# Autodesk Inventor assembly: Functioning elevator (frame)
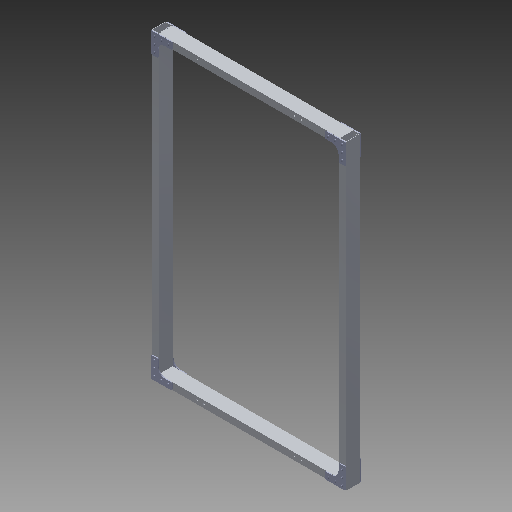
[picture p0: Inventor's stored thumbnail of the model, 512x512]
Saved by Autodesk Inventor 2019 (Build 230136000, 136)
## iProperties
Created: 2019-01-17
Part Number: Functioning elevator (frame)
Document SubType Name: Assembly
Designer: josh
Mass: 2454.62 g
Surface Area: 11117.3 cm^2
Volume: 909.118 cm^3
Density: 2.7 g/cm^3
Author: josh
## Documents named in this file (4)
- D:\Synthesis Robots\Epsilon\Epsilon elavator lift\Functioning elevator (frame).iam
- D:\Synthesis Robots\Epsilon\Epsilon elavator lift\Functioning elevator parts\Example Fixed Tube.ipt
- D:\Synthesis Robots\Epsilon\Epsilon elavator lift\Functioning elevator parts\Example Cross Frame Tube.ipt
- D:\Synthesis Robots\Epsilon\Epsilon elavator lift\Functioning elevator parts\am-3860 90 Gusset with Rivets.iam
## Components (12 placed, 3 different names)
1. Example Fixed Tube:1 — Flush:8, Mate:6, Flush:9, Flush:11, Flush:18, Flush:20, Flush:22, Mate:16
2. Example Fixed Tube:2 — Flush:2, Flush:3, Mate:2, Mate:3, Flush:5, Flush:6, Flush:7, Flush:13, Mate:9, Flush:16, Flush:17, Mate:15
3. Example Cross Frame Tube:1 — Flush:14, Flush:15, Mate:11, Mate:12, Flush:17, Flush:19, Mate:13, Flush:21, Mate:14, Mate:15, Mate:16
4. Example Cross Frame Tube:2 — Mate:1, Mate:2, Flush:4, Mate:4, Flush:8, Flush:10, Mate:7, Flush:12, Mate:8
5. am-3860 90 Gusset with Rivets:1 [sub-assembly] — Flush:13, Flush:14, Mate:9, Mate:11
6. am-3860 90 Gusset with Rivets:2 [sub-assembly] — Flush:15, Flush:16, Mate:12
7. am-3860 90 Gusset with Rivets:3 [sub-assembly] — Flush:18, Flush:21, Flush:22, Mate:14
8. am-3860 90 Gusset with Rivets:4 [sub-assembly] — Flush:19, Flush:20, Mate:13
9. am-3860 90 Gusset with Rivets:5 [sub-assembly] — Flush:3, Flush:6, Flush:7, Mate:4
10. am-3860 90 Gusset with Rivets:6 [sub-assembly] — Mate:1, Flush:2, Flush:4, Mate:3, Flush:5
11. am-3860 90 Gusset with Rivets:7 [sub-assembly] — Mate:6, Flush:9, Flush:10, Mate:7
12. am-3860 90 Gusset with Rivets:8 [sub-assembly] — Flush:11, Flush:12, Mate:8
## Relationships (35: Flush 21, Mate 14)
- Mate:1: Example Cross Frame Tube:2 ↔ am-3860 90 Gusset with Rivets:6
- Flush:2: Example Fixed Tube:2 ↔ am-3860 90 Gusset with Rivets:6
- Flush:3: Example Fixed Tube:2 ↔ am-3860 90 Gusset with Rivets:5
- Mate:2: Example Fixed Tube:2 ↔ Example Cross Frame Tube:2
- Flush:4: Example Cross Frame Tube:2 ↔ am-3860 90 Gusset with Rivets:6
- Mate:3: Example Fixed Tube:2 ↔ am-3860 90 Gusset with Rivets:6
- Flush:5: Example Fixed Tube:2 ↔ am-3860 90 Gusset with Rivets:6
- Flush:6: Example Fixed Tube:2 ↔ am-3860 90 Gusset with Rivets:5
- Flush:7: Example Fixed Tube:2 ↔ am-3860 90 Gusset with Rivets:5
- Mate:4: Example Cross Frame Tube:2 ↔ am-3860 90 Gusset with Rivets:5
- Flush:8: Example Fixed Tube:1 ↔ Example Cross Frame Tube:2
- Mate:6: Example Fixed Tube:1 ↔ am-3860 90 Gusset with Rivets:7
- Flush:9: Example Fixed Tube:1 ↔ am-3860 90 Gusset with Rivets:7
- Flush:10: Example Cross Frame Tube:2 ↔ am-3860 90 Gusset with Rivets:7
- Mate:7: Example Cross Frame Tube:2 ↔ am-3860 90 Gusset with Rivets:7
- Flush:11: Example Fixed Tube:1 ↔ am-3860 90 Gusset with Rivets:8
- Flush:12: Example Cross Frame Tube:2 ↔ am-3860 90 Gusset with Rivets:8
- Mate:8: Example Cross Frame Tube:2 ↔ am-3860 90 Gusset with Rivets:8
- Flush:13: Example Fixed Tube:2 ↔ am-3860 90 Gusset with Rivets:1
- Flush:14: Example Cross Frame Tube:1 ↔ am-3860 90 Gusset with Rivets:1
- Mate:9: Example Fixed Tube:2 ↔ am-3860 90 Gusset with Rivets:1
- Flush:15: Example Cross Frame Tube:1 ↔ am-3860 90 Gusset with Rivets:2
- Flush:16: Example Fixed Tube:2 ↔ am-3860 90 Gusset with Rivets:2
- Mate:11: Example Cross Frame Tube:1 ↔ am-3860 90 Gusset with Rivets:1
- Mate:12: Example Cross Frame Tube:1 ↔ am-3860 90 Gusset with Rivets:2
- Flush:17: Example Fixed Tube:2 ↔ Example Cross Frame Tube:1
- Flush:18: Example Fixed Tube:1 ↔ am-3860 90 Gusset with Rivets:3
- Flush:19: Example Cross Frame Tube:1 ↔ am-3860 90 Gusset with Rivets:4
- Flush:20: Example Fixed Tube:1 ↔ am-3860 90 Gusset with Rivets:4
- Mate:13: Example Cross Frame Tube:1 ↔ am-3860 90 Gusset with Rivets:4
- Flush:21: Example Cross Frame Tube:1 ↔ am-3860 90 Gusset with Rivets:3
- Flush:22: Example Fixed Tube:1 ↔ am-3860 90 Gusset with Rivets:3
- Mate:14: Example Cross Frame Tube:1 ↔ am-3860 90 Gusset with Rivets:3
- Mate:15: Example Fixed Tube:2 ↔ Example Cross Frame Tube:1
- Mate:16: Example Fixed Tube:1 ↔ Example Cross Frame Tube:1
